# Autodesk Inventor assembly: CAM_T8
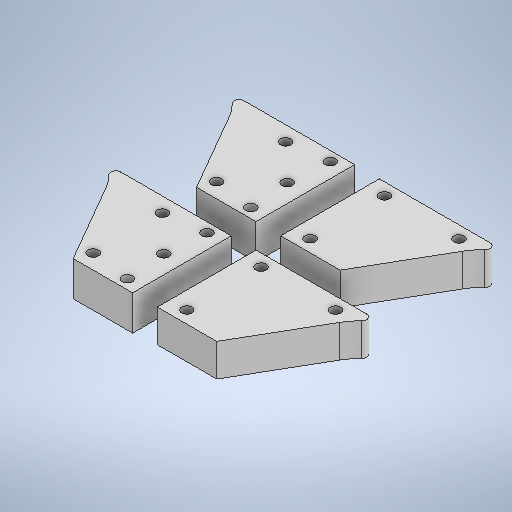
[picture p0: Inventor's stored thumbnail of the model, 512x512]
Saved by Autodesk Inventor 2025.2 (Build 292293000, 293)
## iProperties
Created: 2025-08-10
Part Number: CAM_T8
Document SubType Name: Assembly
Designer: User
Author: User
## Documents named in this file (3)
- C:\Users\User\Documents\The Maverick's Files\College 3-3\로보인 프로젝트\RHp_Humanoid_ver1\Part\Frame\Leg\Left Leg\CAM\CAM_T8.iam
- C:\Users\User\Documents\The Maverick's Files\College 3-3\로보인 프로젝트\RHp_Humanoid_ver1\Part\Frame\Leg\3D_printed_part_non_powered.ipt
- C:\Users\User\Documents\The Maverick's Files\College 3-3\로보인 프로젝트\RHp_Humanoid_ver1\Part\Frame\Leg\3D_printed_part_powered.ipt
## Components (4 placed, 2 different names)
1. 3D_printed_part_non_powered:1 — Flush:1, Flush:2, Flush:3, Flush:4, Mate:1, Flush:5, Mate:2, Flush:6, Flush:7, Flush:8
2. 3D_printed_part_powered:1 — Flush:8, Mate:3, Flush:9
3. 3D_printed_part_non_powered:2 — Flush:4, Mate:1, Flush:5, Mate:3, Flush:9
4. 3D_printed_part_powered:2 — Mate:2, Flush:6, Flush:7
## Relationships (12: Flush 9, Mate 3)
- Flush:1: 3D_printed_part_non_powered:1
- Flush:2: 3D_printed_part_non_powered:1
- Flush:3: 3D_printed_part_non_powered:1
- Flush:4: 3D_printed_part_non_powered:1 ↔ 3D_printed_part_non_powered:2
- Mate:1 (5 mm): 3D_printed_part_non_powered:1 ↔ 3D_printed_part_non_powered:2
- Flush:5: 3D_printed_part_non_powered:1 ↔ 3D_printed_part_non_powered:2
- Mate:2 (5 mm): 3D_printed_part_non_powered:1 ↔ 3D_printed_part_powered:2
- Flush:6: 3D_printed_part_non_powered:1 ↔ 3D_printed_part_powered:2
- Flush:7: 3D_printed_part_non_powered:1 ↔ 3D_printed_part_powered:2
- Flush:8: 3D_printed_part_non_powered:1 ↔ 3D_printed_part_powered:1
- Mate:3 (5 mm): 3D_printed_part_powered:1 ↔ 3D_printed_part_non_powered:2
- Flush:9: 3D_printed_part_powered:1 ↔ 3D_printed_part_non_powered:2
